# Autodesk Inventor assembly: Gearbox_MIR
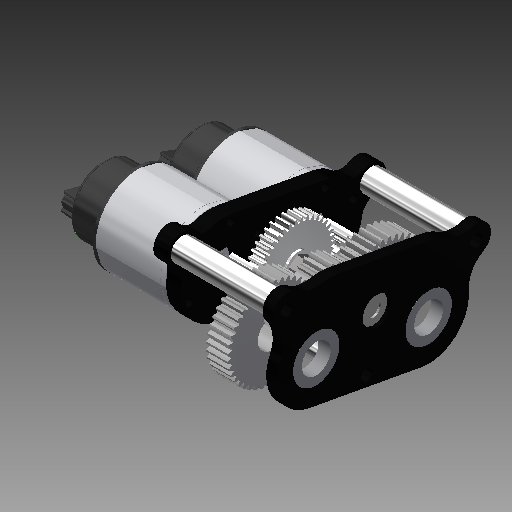
[picture p0: Inventor's stored thumbnail of the model, 512x512]
Saved by Autodesk Inventor 2019.4 (Build 234330000, 330)
## iProperties
Created: 2019-12-11
Part Number: Gearbox_MIR
Document SubType Name: Assembly
Designer: Mark
Author: admin
## Documents named in this file (12)
- C:\Users\Mark\Desktop\7738 Helion Engineering\7738-CAD-prep\Offline CAD\MK3 Gearbox\Gearbox_MIR.iam
- C:\Users\Mark\Desktop\7738 Helion Engineering\7738-CAD-prep\Swerve Module\Falcon_500_Powered_by_Talon_FX_217-6515_MIR1.iam
- C:\Users\Mark\Desktop\7738 Helion Engineering\7738-CAD-prep\WCD\10T_Steel_Spur_Gear_20_DP_12T_Center_Distance_Falcon_Motor_217-6917_MIR1.ipt
- C:\Users\Mark\Desktop\7738 Helion Engineering\7738-CAD-prep\Offline CAD\MK3 Gearbox\40t_Aluminum_Spur_Gear_20_DP_1_2_Hex_Bore_217-2708_MIR.ipt
- C:\Users\Mark\Desktop\7738 Helion Engineering\7738-CAD-prep\Offline CAD\MK3 Gearbox\Gearbox\Design Accelerator\Spur Gears1_MIR.iam
- C:\Users\Mark\Desktop\7738 Helion Engineering\7738-CAD-prep\Offline CAD\MK3 Gearbox\Gearbox Plate 1_MIR.ipt
- C:\Users\Mark\Desktop\7738 Helion Engineering\7738-CAD-prep\Offline CAD\MK3 Gearbox\Gearbox Plate 2_MIR.ipt
- C:\Users\Mark\Desktop\7738 Helion Engineering\7738-CAD-prep\Butterfly drive\F6800Z 10mm ID Flange_MIR2.ipt
- C:\Users\Mark\Desktop\7738 Helion Engineering\7738-CAD-prep\Offline CAD\MK3 Gearbox\Shaft Jr_MIR.ipt
- C:\Users\Mark\Desktop\7738 Helion Engineering\7738-CAD-prep\Offline CAD\F6804_MIR.ipt
- C:\Users\Mark\Desktop\7738 Helion Engineering\7738-CAD-prep\Offline CAD\MK3 Gearbox\Gearbox\Design Accelerator\Spur Gears2_MIR.iam
- C:\Users\Mark\Desktop\7738 Helion Engineering\7738-CAD-prep\Offline CAD\Gearbox Spacer_MIR.ipt
## Components (17 placed, 11 different names)
1. Falcon_500_Powered_by_Talon_FX_217-6515_MIR1:1 [sub-assembly] — Mate:16, Mate:6, Mate:5
2. 10T_Steel_Spur_Gear_20_DP_12T_Center_Distance_Falcon_Motor_217-6917_MIR1:1 — Mate:16, Mate:17
3. 10T_Steel_Spur_Gear_20_DP_12T_Center_Distance_Falcon_Motor_217-6917_MIR1:2 — Mate:18, Mate:15
4. 40t_Aluminum_Spur_Gear_20_DP_1_2_Hex_Bore_217-2708_MIR:1 — Mate:39, Mate:38, Mate:22, Mate:21
5. Spur Gears1_MIR:1 [sub-assembly] — Mate:39, Mate:38, Mate:29, Flush:2
6. Gearbox Plate 1_MIR:1 — Mate:18, Mate:17, Mate:6, Mate:5, Mate:26, Flush:1, Mate:8, Mate:7, Mate:20, Mate:19, Mate:37, Mate:36
7. Gearbox Plate 2_MIR:1 — Mate:26, Flush:1, Mate:10, Mate:9, Mate:12, Mate:11, Mate:14, Mate:13, Mate:33, Mate:32, Mate:35, Mate:34
8. F6800Z 10mm ID Flange_MIR2:1 — Mate:10, Mate:9, Mate:25
9. Shaft Jr_MIR:1 — Mate:25, Mate:24, Mate:23
10. Falcon_500_Powered_by_Talon_FX_217-6515_MIR1:2 [sub-assembly] — Mate:15, Mate:8, Mate:7
11. F6804_MIR:1 — Mate:12, Mate:11, Mate:30
12. F6804_MIR:2 — Mate:29, Mate:14, Mate:13
13. F6800Z 10mm ID Flange_MIR2:2 — Mate:24, Mate:23, Mate:22, Mate:21, Mate:20, Mate:19
14. Spur Gears2_MIR:1 [sub-assembly] — Flush:2, Mate:30
15. Gearbox Spacer_MIR:1 — Mate:33, Mate:32
16. Gearbox Spacer_MIR:2 — Mate:35, Mate:34
17. Gearbox Spacer_MIR:3 — Mate:37, Mate:36
## Relationships (34: Mate 32, Flush 2)
- Mate:16: Falcon_500_Powered_by_Talon_FX_217-6515_MIR1:1 ↔ 10T_Steel_Spur_Gear_20_DP_12T_Center_Distance_Falcon_Motor_217-6917_MIR1:1
- Mate:39 (8 mm): 40t_Aluminum_Spur_Gear_20_DP_1_2_Hex_Bore_217-2708_MIR:1 ↔ Spur Gears1_MIR:1
- Mate:38: 40t_Aluminum_Spur_Gear_20_DP_1_2_Hex_Bore_217-2708_MIR:1 ↔ Spur Gears1_MIR:1
- Mate:18 (1 mm): 10T_Steel_Spur_Gear_20_DP_12T_Center_Distance_Falcon_Motor_217-6917_MIR1:2 ↔ Gearbox Plate 1_MIR:1
- Mate:17 (1 mm): 10T_Steel_Spur_Gear_20_DP_12T_Center_Distance_Falcon_Motor_217-6917_MIR1:1 ↔ Gearbox Plate 1_MIR:1
- Mate:6: Falcon_500_Powered_by_Talon_FX_217-6515_MIR1:1 ↔ Gearbox Plate 1_MIR:1
- Mate:5: Falcon_500_Powered_by_Talon_FX_217-6515_MIR1:1 ↔ Gearbox Plate 1_MIR:1
- Mate:26 (65 mm): Gearbox Plate 1_MIR:1 ↔ Gearbox Plate 2_MIR:1
- Flush:1: Gearbox Plate 1_MIR:1 ↔ Gearbox Plate 2_MIR:1
- Mate:10 (0.1 mm): Gearbox Plate 2_MIR:1 ↔ F6800Z 10mm ID Flange_MIR2:1
- Mate:9: Gearbox Plate 2_MIR:1 ↔ F6800Z 10mm ID Flange_MIR2:1
- Mate:25: F6800Z 10mm ID Flange_MIR2:1 ↔ Shaft Jr_MIR:1
- Mate:15: 10T_Steel_Spur_Gear_20_DP_12T_Center_Distance_Falcon_Motor_217-6917_MIR1:2 ↔ Falcon_500_Powered_by_Talon_FX_217-6515_MIR1:2
- Mate:8: Gearbox Plate 1_MIR:1 ↔ Falcon_500_Powered_by_Talon_FX_217-6515_MIR1:2
- Mate:7: Gearbox Plate 1_MIR:1 ↔ Falcon_500_Powered_by_Talon_FX_217-6515_MIR1:2
- Mate:12: Gearbox Plate 2_MIR:1 ↔ F6804_MIR:1
- Mate:11 (0.1 mm): Gearbox Plate 2_MIR:1 ↔ F6804_MIR:1
- Mate:29: Spur Gears1_MIR:1 ↔ F6804_MIR:2
- Mate:14: Gearbox Plate 2_MIR:1 ↔ F6804_MIR:2
- Mate:13 (0.1 mm): Gearbox Plate 2_MIR:1 ↔ F6804_MIR:2
- Mate:24: Shaft Jr_MIR:1 ↔ F6800Z 10mm ID Flange_MIR2:2
- Mate:23 (0.1 mm): Shaft Jr_MIR:1 ↔ F6800Z 10mm ID Flange_MIR2:2
- Mate:22: 40t_Aluminum_Spur_Gear_20_DP_1_2_Hex_Bore_217-2708_MIR:1 ↔ F6800Z 10mm ID Flange_MIR2:2
- Mate:21 (5 mm): 40t_Aluminum_Spur_Gear_20_DP_1_2_Hex_Bore_217-2708_MIR:1 ↔ F6800Z 10mm ID Flange_MIR2:2
- Mate:20: Gearbox Plate 1_MIR:1 ↔ F6800Z 10mm ID Flange_MIR2:2
- Mate:19 (0.1 mm): Gearbox Plate 1_MIR:1 ↔ F6800Z 10mm ID Flange_MIR2:2
- Flush:2: Spur Gears1_MIR:1 ↔ Spur Gears2_MIR:1
- Mate:30: F6804_MIR:1 ↔ Spur Gears2_MIR:1
- Mate:33 (0.2 mm): Gearbox Plate 2_MIR:1 ↔ Gearbox Spacer_MIR:1
- Mate:32: Gearbox Plate 2_MIR:1 ↔ Gearbox Spacer_MIR:1
- Mate:35 (0.2 mm): Gearbox Plate 2_MIR:1 ↔ Gearbox Spacer_MIR:2
- Mate:34: Gearbox Plate 2_MIR:1 ↔ Gearbox Spacer_MIR:2
- Mate:37 (0.2 mm): Gearbox Plate 1_MIR:1 ↔ Gearbox Spacer_MIR:3
- Mate:36: Gearbox Plate 1_MIR:1 ↔ Gearbox Spacer_MIR:3
